# Autodesk Inventor assembly: assembly
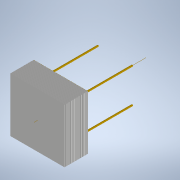
[picture p0: Inventor's stored thumbnail of the model, 180x180]
Saved by Autodesk Inventor 2021 (Build 250183000, 183)
## iProperties
Created: 2020-07-29
Part Number: assembly
Document SubType Name: Assembly
Designer: aydan
Author: aydan
## Documents named in this file (3)
- C:\Users\aydan\Documents\Inventor\Garcia_Lab\CAD_Models\assembly.iam
- C:\Users\aydan\Documents\Inventor\Garcia_Lab\CAD_Models\electrode.ipt
- C:\Users\aydan\Documents\Inventor\Garcia_Lab\CAD_Models\electrode_holder.ipt
## Components (102 placed, 2 different names)
1. electrode:1
2. electrode:2
3. electrode:3
4. electrode:4
5. electrode:5
6. electrode:6
7. electrode:7
8. electrode:8
9. electrode:9
10. electrode:10
11. electrode:11
12. electrode:12
13. electrode:13
14. electrode:14
15. electrode:15
16. electrode:16
17. electrode:17
18. electrode:18
19. electrode:19
20. electrode:20
21. electrode:21
22. electrode:22
23. electrode:23
24. electrode:24
25. electrode:25
26. electrode:26
27. electrode:27
28. electrode:28
29. electrode:29
30. electrode:30
31. electrode:31
32. electrode:32
33. electrode:33
34. electrode:34
35. electrode:35
36. electrode:36
37. electrode:37
38. electrode:38
39. electrode:39
40. electrode:40
41. electrode:41
42. electrode:42
43. electrode:43
44. electrode:44
45. electrode:45
46. electrode:46
47. electrode:47
48. electrode:48
49. electrode:49
50. electrode:50
51. electrode:51
52. electrode:52
53. electrode:53
54. electrode:54
55. electrode:55
56. electrode:56
57. electrode:57
58. electrode:58
59. electrode:59
60. electrode:60
61. electrode:61
62. electrode:62
63. electrode:63
64. electrode:64
65. electrode:65
66. electrode:66
67. electrode:67
68. electrode:68
69. electrode:69
70. electrode:70
71. electrode:71
72. electrode:72
73. electrode:73
74. electrode:74
75. electrode:75
76. electrode:76
77. electrode:77
78. electrode:78
79. electrode:79
80. electrode:80
81. electrode:81
82. electrode:82
83. electrode:83
84. electrode:84
85. electrode:85
86. electrode:86
87. electrode:87
88. electrode:88
89. electrode:89
90. electrode:90
91. electrode:91
92. electrode:92
93. electrode:93
94. electrode:94
95. electrode:95
96. electrode:96
97. electrode:97
98. electrode:98
99. electrode:99
100. electrode:100
101. electrode:101 — Mate:5
102. electrode_holder:1 — Mate:1, Mate:5
## Relationships (6: Mate 5, Flush 1)
- Flush:1
- Mate:1: electrode_holder:1
- Mate:2
- Mate:3
- Mate:4
- Mate:5: electrode:101 ↔ electrode_holder:1
